# Autodesk Inventor assembly: M - Rail 1
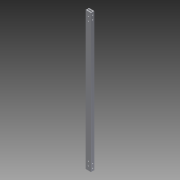
[picture p0: Inventor's stored thumbnail of the model, 180x180]
Saved by Autodesk Inventor 2013 (Build 170138000, 138)
## iProperties
Created: 2013-02-16
Part Number: M - Rail 1
Document SubType Name: Assembly
Designer: Moses
Mass: 499.27 g
Surface Area: 1553.87 cm^2
Volume: 184.232 cm^3
Density: 2.71 g/cm^3
Author: Moses
## Documents named in this file (9)
- C:\Users\Arpan\Documents\GitHub\frc2013CAD\M-Climber\M - Rail 1.iam
- C:\Users\Arpan\Documents\GitHub\frc2013CAD\M-Climber\M - 26 inch rail.ipt
- C:\Users\Arpan\Documents\GitHub\frc2013CAD\M-Climber\M - 26 inch rail surface.ipt
- C:\Users\Arpan\Documents\GitHub\frc2013CAD\M-Climber\M - Rail 1\AIP\FEA\aln6c11b4.fins
- C:\Users\Arpan\Documents\GitHub\frc2013CAD\M-Climber\M - Rail 1\AIP\FEA\aln6c11b4.fsat
- C:\Users\Arpan\Documents\GitHub\frc2013CAD\M-Climber\M - Rail 1\AIP\FEA\aln6c11b4.ftes
- C:\Users\Arpan\Documents\GitHub\frc2013CAD\M-Climber\M - Rail 1\AIP\FEA\aln6c11b4.fwiz
- C:\Users\Arpan\Documents\GitHub\frc2013CAD\M-Climber\M - Rail 1\AIP\FEA\aln6c11cw.fmsh
- C:\Users\Arpan\Documents\GitHub\frc2013CAD\M-Climber\M - Rail 1\AIP\FEA\aln6c11cx.fres
## Components (3 placed, 2 different names)
1. M - 26 inch rail:1 — Mate:1, Mate:2, Flush:1, Mate:3, Flush:2, Flush:3
2. M - 26 inch rail surface:1 — Mate:1, Mate:2, Flush:1
3. M - 26 inch rail surface:2 — Mate:3, Flush:2, Flush:3
## Relationships (6: Mate 3, Flush 3)
- Mate:1: M - 26 inch rail:1 ↔ M - 26 inch rail surface:1
- Mate:2: M - 26 inch rail:1 ↔ M - 26 inch rail surface:1
- Flush:1: M - 26 inch rail:1 ↔ M - 26 inch rail surface:1
- Mate:3: M - 26 inch rail:1 ↔ M - 26 inch rail surface:2
- Flush:2: M - 26 inch rail:1 ↔ M - 26 inch rail surface:2
- Flush:3: M - 26 inch rail:1 ↔ M - 26 inch rail surface:2
## Named parameters: sa_0 = 0, sa_1 = 0, sa_2 = 667233, sa_3 = 0, sa_4 = 0, sa_5 = -667233
note: some values were not read from the file. Shown as the stored number, unit unknown: "sa_0", "sa_1", "sa_2", "sa_3", "sa_4", "sa_5".
